# Autodesk Inventor assembly: mecanum wheel MIR
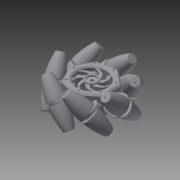
[picture p0: Inventor's stored thumbnail of the model, 180x180]
Saved by Autodesk Inventor 2015 (Build 190159000, 159)
## iProperties
Created: 2016-09-13
Part Number: mecanum wheel MIR
Document SubType Name: Assembly
Designer: 294591
Title: 276-1447.STEP
Description: STEP AP203
Creation Date: 2011-11-15
Sending System: SolidWorks 2010
Preprocessor: SwSTEP 2.0
Author: 294591
## Documents named in this file (8)
- \\stushare\home\294591\Documents\Inventor\robotics\Imported Components\276-1447\mecanum wheel MIR.iam
- \\stushare\home\294591\Documents\Inventor\robotics\Imported Components\276-1447\WHEEL_MIR.ipt
- \\stushare\home\294591\Documents\Inventor\robotics\Imported Components\276-1447\WASHER_MIR.ipt
- \\stushare\home\294591\Documents\Inventor\robotics\Imported Components\276-1447\BRACKET-R_MIR.ipt
- \\stushare\home\294591\Documents\Inventor\robotics\Imported Components\276-1447\SMALL-WHEEL-HUB_MIR.ipt
- \\stushare\home\294591\Documents\Inventor\robotics\Imported Components\276-1447\PIN_MIR.ipt
- \\stushare\home\294591\Documents\Inventor\robotics\Imported Components\276-1447\WHEEL-HUB-IN-R_MIR.ipt
- \\stushare\home\294591\Documents\Inventor\robotics\Imported Components\276-1447\WHEEL-HUB-OUT-R_MIR.ipt
## Components (58 placed, 7 different names)
1. WHEEL_MIR:1
2. WASHER_MIR:1
3. BRACKET-R_MIR:1
4. SMALL-WHEEL-HUB_MIR:1
5. PIN_MIR:1
6. WHEEL_MIR:2
7. WASHER_MIR:2
8. WHEEL_MIR:3
9. WASHER_MIR:3
10. BRACKET-R_MIR:2
11. PIN_MIR:2
12. WHEEL_MIR:4
13. WASHER_MIR:4
14. WHEEL_MIR:5
15. WASHER_MIR:5
16. BRACKET-R_MIR:3
17. BRACKET-R_MIR:4
18. SMALL-WHEEL-HUB_MIR:2
19. WHEEL_MIR:6
20. WASHER_MIR:6
21. WHEEL_MIR:7
22. WASHER_MIR:7
23. BRACKET-R_MIR:5
24. SMALL-WHEEL-HUB_MIR:3
25. WHEEL_MIR:8
26. WASHER_MIR:8
27. SMALL-WHEEL-HUB_MIR:4
28. SMALL-WHEEL-HUB_MIR:5
29. PIN_MIR:3
30. WASHER_MIR:9
31. BRACKET-R_MIR:6
32. SMALL-WHEEL-HUB_MIR:6
33. SMALL-WHEEL-HUB_MIR:7
34. WHEEL_MIR:9
35. WASHER_MIR:10
36. SMALL-WHEEL-HUB_MIR:8
37. PIN_MIR:4
38. WASHER_MIR:11
39. BRACKET-R_MIR:7
40. SMALL-WHEEL-HUB_MIR:9
41. WHEEL_MIR:10
42. WASHER_MIR:12
43. PIN_MIR:5
44. WHEEL-HUB-IN-R_MIR:1 — Flush:1
45. SMALL-WHEEL-HUB_MIR:10
46. SMALL-WHEEL-HUB_MIR:11
47. SMALL-WHEEL-HUB_MIR:12
48. WHEEL_MIR:11
49. WASHER_MIR:13
50. SMALL-WHEEL-HUB_MIR:13
51. PIN_MIR:6
52. WHEEL_MIR:12
53. SMALL-WHEEL-HUB_MIR:14
54. WHEEL_MIR:13
55. WASHER_MIR:14
56. WHEEL-HUB-OUT-R_MIR:1
57. PIN_MIR:7
58. WHEEL_MIR:14
## Relationships (1: Flush 1)
- Flush:1 (53.975 mm): WHEEL-HUB-IN-R_MIR:1
